# Autodesk Inventor assembly: Biela Completa
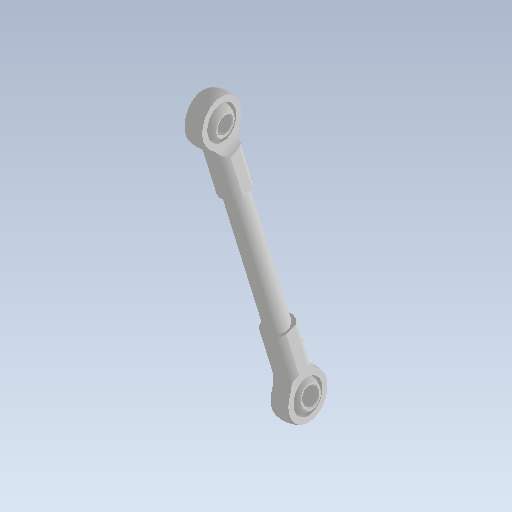
[picture p0: Inventor's stored thumbnail of the model, 512x512]
Saved by Autodesk Inventor 2021 (Build 250183000, 183)
## iProperties
Created: 2021-06-19
Part Number: Biela Completa
Document SubType Name: Assembly
Designer: Andrés Holguín
Author: Andrés Holguín
## Documents named in this file (3)
- C:\Users\andre\Documents\GitHub\Dis.-Mecatronico-E6\inventor proyecto\Motores y reductores\Biela Completa.iam
- C:\Users\andre\Documents\GitHub\Dis.-Mecatronico-E6\inventor proyecto\Motores y reductores\Eje Biela.ipt
- C:\Users\andre\Documents\GitHub\Dis.-Mecatronico-E6\inventor proyecto\Motores y reductores\rotula.iam
## Components (3 placed, 2 different names)
1. Eje Biela:1 — Rigid:1, Rigid:2
2. rotula:1 [sub-assembly] — Rigid:1
3. rotula:2 [sub-assembly] — Rigid:2
## Relationships (2: WeldJoint 2)
- Rigid:1 [WeldJoint]: Eje Biela:1 ↔ rotula:1
- Rigid:2 [WeldJoint]: Eje Biela:1 ↔ rotula:2
